# Autodesk Inventor assembly: Муфта 30мм
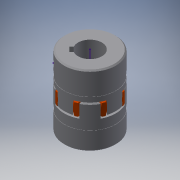
[picture p0: Inventor's stored thumbnail of the model, 180x180]
Saved by Autodesk Inventor 2016 (Build 200138000, 138)
## iProperties
Created: 2021-04-30
Part Number: Муфта 30мм
Material: Типовые
Document SubType Name: Assembly
Designer: Лол
Author: Лол
## Documents named in this file (3)
- C:\Users\Лол\Documents\Inventor\course_work\Муфта 30мм.iam
- C:\Users\Лол\Documents\Inventor\course_work\Муфта резинка 30мм.ipt
- C:\Users\Лол\Documents\Inventor\course_work\Муфта железка 30мм.ipt
## Components (3 placed, 2 different names)
1. Муфта железка 30мм:1 — Совмещение:1, Совмещение:2, Совмещение:4, Угол:1
2. Муфта железка 30мм:2 — Совмещение:3, Совмещение:4, Угол:1, Угол:2
3. Муфта резинка 30мм:1 — Совмещение:1, Совмещение:2, Совмещение:3, Угол:2
## Relationships (6: Mate 4, Angle 2)
- Совмещение:1 [Mate]: Муфта железка 30мм:1 ↔ Муфта резинка 30мм:1
- Совмещение:2 [Mate]: Муфта железка 30мм:1 ↔ Муфта резинка 30мм:1
- Совмещение:3 [Mate]: Муфта железка 30мм:2 ↔ Муфта резинка 30мм:1
- Совмещение:4 [Mate]: Муфта железка 30мм:1 ↔ Муфта железка 30мм:2
- Угол:1 [Angle] (45 deg): Муфта железка 30мм:1 ↔ Муфта железка 30мм:2
- Угол:2 [Angle] (22.5 deg): Муфта железка 30мм:2 ↔ Муфта резинка 30мм:1
